# Autodesk Inventor assembly: 装配-刀
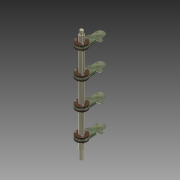
[picture p0: Inventor's stored thumbnail of the model, 180x180]
Saved by Autodesk Inventor 2015 (Build 190159000, 159)
## iProperties
Created: 2017-05-24
Part Number: 装配-刀
Document SubType Name: Assembly
Designer: Administrator
Author: Administrator
## Documents named in this file (6)
- C:\Users\Administrator\Desktop\毕设改\装配-刀.iam
- C:\Users\Administrator\Desktop\毕设改\刀.ipt
- C:\Users\Administrator\Desktop\毕设改\刀夹片.ipt
- C:\Users\Administrator\Desktop\毕设改\刀夹片紧固螺帽.ipt
- C:\Users\Administrator\Desktop\毕设改\刀夹片紧固螺丝.ipt
- C:\Users\Administrator\Desktop\毕设改\刀轴.ipt
## Components (37 placed, 5 different names)
1. 刀轴:1 — 插入:1, 配合:1
2. 刀:1 — 插入:1, 配合:1, 插入:2, 插入:3, 插入:4, 插入:5
3. 刀夹片:1 — 插入:2, 插入:3, 插入:7
4. 刀夹片:2 — 插入:4, 插入:5, 插入:6
5. 刀:2
6. 刀夹片:3
7. 刀夹片:4
8. 刀:3
9. 刀夹片:5
10. 刀夹片:6
11. 刀:4
12. 刀夹片:7
13. 刀夹片:8
14. 刀夹片紧固螺帽:1 — 插入:7
15. 刀夹片紧固螺丝:1 — 插入:6
16. 刀夹片紧固螺帽:2
17. 刀夹片紧固螺丝:2
18. 刀夹片紧固螺帽:3
19. 刀夹片紧固螺丝:3
20. 刀夹片紧固螺帽:4
21. 刀夹片紧固螺丝:4
22. 刀夹片紧固螺帽:5
23. 刀夹片紧固螺丝:5
24. 刀夹片紧固螺帽:6
25. 刀夹片紧固螺丝:6
26. 刀夹片紧固螺帽:7
27. 刀夹片紧固螺丝:7
28. 刀夹片紧固螺帽:8
29. 刀夹片紧固螺丝:8
30. 刀夹片紧固螺帽:9
31. 刀夹片紧固螺丝:9
32. 刀夹片紧固螺帽:10
33. 刀夹片紧固螺丝:10
34. 刀夹片紧固螺帽:11
35. 刀夹片紧固螺丝:11
36. 刀夹片紧固螺帽:12
37. 刀夹片紧固螺丝:12
## Component patterns: (4 elements, first: 刀:1 + 刀夹片:1 + 刀夹片:2), (3 elements, first: 刀夹片紧固螺帽:1 + 刀夹片紧固螺丝:1), 零部件阵列 1:2 (3 elements), 零部件阵列 1:3 (3 elements), 零部件阵列 1:4 (3 elements)
## Relationships (8: Insert 7, Mate 1)
- 插入:1 [Insert]: 刀轴:1 ↔ 刀:1
- 配合:1 [Mate]: 刀轴:1 ↔ 刀:1
- 插入:2 [Insert]: 刀:1 ↔ 刀夹片:1
- 插入:3 [Insert]: 刀:1 ↔ 刀夹片:1
- 插入:4 [Insert]: 刀:1 ↔ 刀夹片:2
- 插入:5 [Insert]: 刀:1 ↔ 刀夹片:2
- 插入:6 [Insert]: 刀夹片:2 ↔ 刀夹片紧固螺丝:1
- 插入:7 [Insert]: 刀夹片:1 ↔ 刀夹片紧固螺帽:1
